# Autodesk Inventor assembly: AL_plate_600x460x2t_door
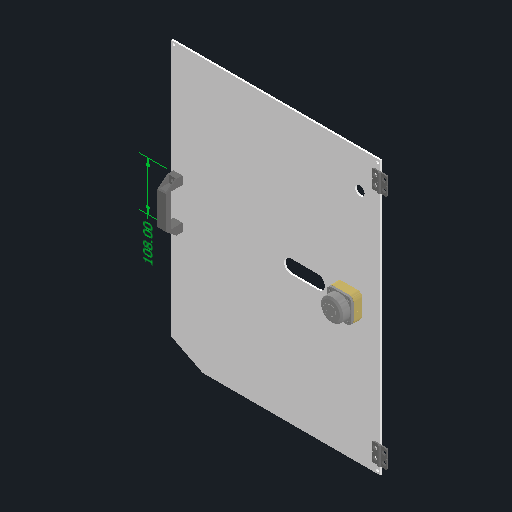
[picture p0: Inventor's stored thumbnail of the model, 512x512]
Saved by Autodesk Inventor 2026.2 (Build 302298010, 298A)
## iProperties
Created: 2026-06-10
Part Number: AL_plate_600x460x2t_door
Document SubType Name: Assembly
Designer: dalbi
Author: dalbi
## Documents named in this file (5)
- C:\Users\User\Desktop\트리보 관련 자료\최종 설계 파일(조립시 참고할 파일)\Acryil_door_600x460x2t.iam
- C:\Users\User\Desktop\트리보 관련 자료\최종 설계 파일(조립시 참고할 파일)\Acryil_Plate_Outer_600X460X4t_Cover.ipt
- C:\Users\User\Desktop\트리보 관련 자료\최종 설계 파일(조립시 참고할 파일)\Handle.ipt
- C:\Users\User\Desktop\트리보 관련 자료\최종 설계 파일(조립시 참고할 파일)\Plastic_Hinge.ipt
- C:\Users\User\Desktop\트리보 관련 자료\최종 설계 파일(조립시 참고할 파일)\Lidar.ipt
## Components (7 placed, 4 different names)
1. Acryil_Plate_Outer_600X460X4t_Cover:1 — 메이트:1, 메이트:2, 플러쉬:1, 메이트:3, 메이트:4, 메이트:7, 메이트:8, 메이트:9, 메이트:11, 메이트:12, 플러쉬:6, 플러쉬:7, 플러쉬:8
2. Handle:1 — 메이트:1, 플러쉬:1, 플러쉬:8
3. Plastic_Hinge:1 — 메이트:2, 메이트:3, 메이트:5, 플러쉬:4
4. Plastic_Hinge:2 — 메이트:4, 메이트:5, 플러쉬:4, 플러쉬:6
5. Plastic_Hinge:3 — 메이트:7, 메이트:8, 메이트:10, 플러쉬:7
6. Plastic_Hinge:4 — 메이트:10, 메이트:11
7. Lidar:1 — 메이트:9, 메이트:12
## Relationships (18: Mate 12, Flush 6)
- 메이트:1 [Mate]: Acryil_Plate_Outer_600X460X4t_Cover:1 ↔ Handle:1
- 메이트:2 [Mate]: Acryil_Plate_Outer_600X460X4t_Cover:1 ↔ Plastic_Hinge:1
- 플러쉬:1 [Flush] (246 mm): Acryil_Plate_Outer_600X460X4t_Cover:1 ↔ Handle:1
- 메이트:3 [Mate] (-15 mm): Acryil_Plate_Outer_600X460X4t_Cover:1 ↔ Plastic_Hinge:1
- 메이트:4 [Mate]: Acryil_Plate_Outer_600X460X4t_Cover:1 ↔ Plastic_Hinge:2
- 메이트:5 [Mate]: Plastic_Hinge:1 ↔ Plastic_Hinge:2
- 플러쉬:4 [Flush]: Plastic_Hinge:1 ↔ Plastic_Hinge:2
- [Mate]: Plastic_Hinge:3 ↔ Plastic_Hinge:4
- [Flush]: Plastic_Hinge:3 ↔ Plastic_Hinge:4
- 메이트:7 [Mate]: Acryil_Plate_Outer_600X460X4t_Cover:1 ↔ Plastic_Hinge:3
- 메이트:8 [Mate] (-15 mm): Acryil_Plate_Outer_600X460X4t_Cover:1 ↔ Plastic_Hinge:3
- 메이트:9 [Mate]: Acryil_Plate_Outer_600X460X4t_Cover:1 ↔ Lidar:1
- 메이트:10 [Mate]: Plastic_Hinge:3 ↔ Plastic_Hinge:4
- 메이트:11 [Mate]: Acryil_Plate_Outer_600X460X4t_Cover:1 ↔ Plastic_Hinge:4
- 메이트:12 [Mate]: Acryil_Plate_Outer_600X460X4t_Cover:1 ↔ Lidar:1
- 플러쉬:6 [Flush] (20 mm): Acryil_Plate_Outer_600X460X4t_Cover:1 ↔ Plastic_Hinge:2
- 플러쉬:7 [Flush] (20 mm): Acryil_Plate_Outer_600X460X4t_Cover:1 ↔ Plastic_Hinge:3
- 플러쉬:8 [Flush] (5 mm): Acryil_Plate_Outer_600X460X4t_Cover:1 ↔ Handle:1
## Named parameters: d13_d11 = 0 mm, d14_d12 = 0 mm
